# Autodesk Inventor assembly: 3532_20210408113519_4080L + cover
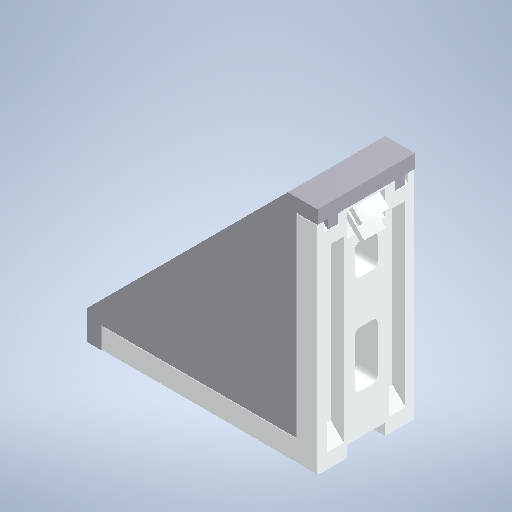
[picture p0: Inventor's stored thumbnail of the model, 512x512]
Saved by Autodesk Inventor 2025.3 (Build 293356000, 356)
## iProperties
Created: 2021-04-08
Part Number: 3532_20210408113519_4080L + cover
Description: STEP AP214
Document SubType Name: Assembly
Designer: louis
Sending System: SolidWorks 2018
Preprocessor: SwSTEP 2.0
Title: 4080L + cover.STEP
Revision Number: ANY
## Documents named in this file (3)
- C:\Users\louis\OneDrive\Desktop\R_Trident\02_CAD\01_Standard_Parts\03_FRM_Fastener\4080L\A_4080L.iam
- C:\Users\louis\OneDrive\Desktop\R_Trident\02_CAD\01_Standard_Parts\03_FRM_Fastener\4080L\4080L+Cover.ipt
- C:\Users\louis\OneDrive\Desktop\R_Trident\02_CAD\01_Standard_Parts\03_FRM_Fastener\4080L\4080L cover.ipt
## Components (2 placed, 2 different names)
1. 4080L+Cover_1 — Flush:1, Flush:2, Flush:3
2. 4080L cover_2 — Flush:1, Flush:2, Flush:3
## Relationships (3: Flush 3)
- Flush:1: 4080L+Cover_1 ↔ 4080L cover_2
- Flush:2: 4080L+Cover_1 ↔ 4080L cover_2
- Flush:3: 4080L+Cover_1 ↔ 4080L cover_2
